# Autodesk Inventor assembly: Bolt Nut Washer assem_MIR
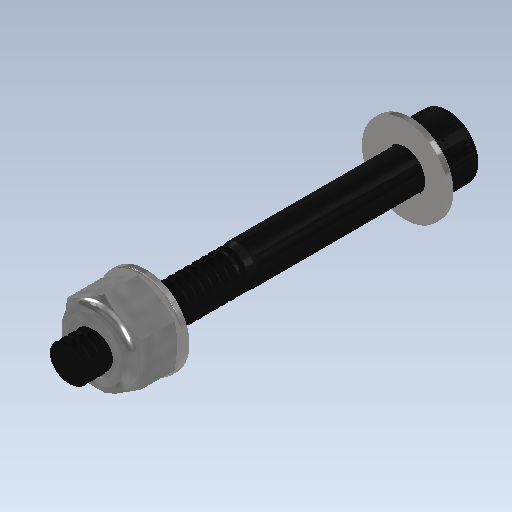
[picture p0: Inventor's stored thumbnail of the model, 512x512]
Saved by Autodesk Inventor 2023 (Build 270158000, 158)
## iProperties
Created: 2023-04-07
Part Number: Bolt Nut Washer assem_MIR
Document SubType Name: Assembly
Designer: Dave
Author: Dave
## Documents named in this file (4)
- C:\Users\Dave\Documents\GitHub\BehrendURCMechanical\CAD\Chassis V3\Bolt Nut Washer assem_MIR.iam
- C:\Users\Dave\Documents\GitHub\BehrendURCMechanical\CAD\Chassis V3\90107A011_316 Stainless Steel Washer_MIR.ipt
- C:\Users\Dave\Documents\GitHub\BehrendURCMechanical\CAD\Chassis V3\91251A252_Black-Oxide Alloy Steel Socket Head Screw_MIR.ipt
- C:\Users\Dave\Documents\GitHub\BehrendURCMechanical\CAD\Chassis V3\91831A011_18-8 Stainless Steel Nylon-Insert Locknut_MIR.ipt
## Components (4 placed, 3 different names)
1. 90107A011_316 Stainless Steel Washer_MIR:1 — Mate:2, Insert:2, Mate:1
2. 91251A252_Black-Oxide Alloy Steel Socket Head Screw_MIR:1 — Mate:2, Insert:1
3. 91831A011_18-8 Stainless Steel Nylon-Insert Locknut_MIR:1 — Insert:2
4. 90107A011_316 Stainless Steel Washer_MIR:2 — Mate:1, Insert:1
## Relationships (4: Mate 2, Insert 2)
- Mate:2: 90107A011_316 Stainless Steel Washer_MIR:1 ↔ 91251A252_Black-Oxide Alloy Steel Socket Head Screw_MIR:1
- Insert:2: 90107A011_316 Stainless Steel Washer_MIR:1 ↔ 91831A011_18-8 Stainless Steel Nylon-Insert Locknut_MIR:1
- Mate:1 (33.3629 mm): 90107A011_316 Stainless Steel Washer_MIR:1 ↔ 90107A011_316 Stainless Steel Washer_MIR:2
- Insert:1: 91251A252_Black-Oxide Alloy Steel Socket Head Screw_MIR:1 ↔ 90107A011_316 Stainless Steel Washer_MIR:2
